# Autodesk Inventor assembly: circuittmp
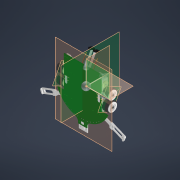
[picture p0: Inventor's stored thumbnail of the model, 180x180]
Saved by Autodesk Inventor 2022 (Build 260153000, 153)
## iProperties
Created: 2022-02-06
Part Number: circuittmp
Document SubType Name: Assembly
Designer: shiokaze
Author: shiokaze
## Documents named in this file (7)
- C:\Users\shiok\Documents\GitHub\murakumo\inventor\circuittmp.iam
- C:\Users\shiok\Documents\GitHub\murakumo\circuit\kicad\Step\Main.iam
- C:\Users\shiok\Documents\GitHub\murakumo\inventor\Motor_MIR.iam
- C:\Users\shiok\Documents\GitHub\murakumo\inventor\jump.ipt
- C:\Users\shiok\Documents\GitHub\murakumo\inventor\SideSensorMount.ipt
- C:\Users\shiok\Documents\GitHub\murakumo\inventor\battery.ipt
- C:\Users\shiok\Documents\GitHub\murakumo\inventor\Motor_MIR_MIR.iam
## Components (7 placed, 6 different names)
1. Main:1 [sub-assembly] — メイト:1, メイト:2, メイト:3, メイト:10, 挿入:1, メイト:13, メイト:14, メイト:15, 角度:1, メイト:18, 挿入:2, メイト:25
2. Motor_MIR:1 [sub-assembly] — メイト:1, メイト:2, メイト:3, メイト:26
3. jump:1 — メイト:13, メイト:14, メイト:15
4. SideSensorMount:1 — メイト:10, 挿入:1
5. battery:1 — メイト:18, メイト:19, メイト:20
6. SideSensorMount:2 — 挿入:2
7. Motor_MIR_MIR:1 [sub-assembly] — フラッシュ:2
## Relationships (17: Mate 13, Insert 2, Angle 1, Flush 1)
- メイト:1 [Mate]: Main:1 ↔ Motor_MIR:1
- メイト:2 [Mate]: Main:1 ↔ Motor_MIR:1
- メイト:3 [Mate]: Main:1 ↔ Motor_MIR:1
- メイト:10 [Mate]: Main:1 ↔ SideSensorMount:1
- 挿入:1 [Insert]: Main:1 ↔ SideSensorMount:1
- メイト:13 [Mate]: Main:1 ↔ jump:1
- メイト:14 [Mate]: Main:1 ↔ jump:1
- メイト:15 [Mate]: Main:1 ↔ jump:1
- 角度:1 [Angle] (0 deg): Main:1
- メイト:18 [Mate]: Main:1 ↔ battery:1
- メイト:19 [Mate]: battery:1
- メイト:20 [Mate]: battery:1
- 挿入:2 [Insert]: Main:1 ↔ SideSensorMount:2
- メイト:24 [Mate]
- メイト:25 [Mate]: Main:1
- メイト:26 [Mate]: Motor_MIR:1
- フラッシュ:2 [Flush]: Motor_MIR_MIR:1
